# Autodesk Inventor assembly: Plattenzusammensetzung
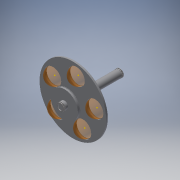
[picture p0: Inventor's stored thumbnail of the model, 180x180]
Saved by Autodesk Inventor 2016 (Build 200138000, 138)
## iProperties
Created: 2017-10-13
Part Number: Plattenzusammensetzung
Material: Generisch
Document SubType Name: Assembly
Designer: Dominik
Author: Dominik
## Documents named in this file (6)
- C:\Users\Dominik\Desktop\Diplomarbeit\Inverntorskizzen\Plattenzusammensetzung.iam
- C:\Users\Dominik\Desktop\Diplomarbeit\Inverntorskizzen\Antriebsscheibe.ipt
- C:\Users\Dominik\Desktop\Diplomarbeit\Inverntorskizzen\Drehplatte_Rahmenvorrrichtung.ipt
- C:\Users\Dominik\Desktop\Diplomarbeit\Inverntorskizzen\Futterschüssel_innen.ipt
- C:\Users\Dominik\Desktop\Diplomarbeit\Inverntorskizzen\Welle.ipt
- C:\Users\Dominik\Documents\Inventor\Content Center Files\R2016\de-DE\DIN 711\DIN 711 - 511 06 - 30 x 47 x 11.ipt
## Components (10 placed, 5 different names)
1. Antriebsscheibe:1 — Passend:2
2. Drehplatte_Rahmenvorrrichtung:1 — Passend:1, Passend:3, Passend:4, Passend:5, Passend:6, Passend:7, Passend:8, Passend:9, Passend:10, Passend:11, Passend:12
3. Futterschüssel_innen:1 — Passend:3, Passend:4
4. Welle:1 — Passend:1, Passend:2, Passend:13, Passend:14, Passend:15, Passend:16
5. Futterschüssel_innen:2 — Passend:5, Passend:6
6. Futterschüssel_innen:3 — Passend:11, Passend:12
7. Futterschüssel_innen:4 — Passend:9, Passend:10
8. Futterschüssel_innen:5 — Passend:7, Passend:8
9. DIN 711 511 06 - 30 x 47 x 11:1 — Passend:13, Passend:16
10. DIN 711 511 06 - 30 x 47 x 11:2 — Passend:14, Passend:15
## Relationships (16: Mate 16)
- Passend:1 [Mate]: Drehplatte_Rahmenvorrrichtung:1 ↔ Welle:1
- Passend:2 [Mate]: Antriebsscheibe:1 ↔ Welle:1
- Passend:3 [Mate]: Drehplatte_Rahmenvorrrichtung:1 ↔ Futterschüssel_innen:1
- Passend:4 [Mate]: Drehplatte_Rahmenvorrrichtung:1 ↔ Futterschüssel_innen:1
- Passend:5 [Mate]: Drehplatte_Rahmenvorrrichtung:1 ↔ Futterschüssel_innen:2
- Passend:6 [Mate]: Drehplatte_Rahmenvorrrichtung:1 ↔ Futterschüssel_innen:2
- Passend:7 [Mate]: Drehplatte_Rahmenvorrrichtung:1 ↔ Futterschüssel_innen:5
- Passend:8 [Mate]: Drehplatte_Rahmenvorrrichtung:1 ↔ Futterschüssel_innen:5
- Passend:9 [Mate]: Drehplatte_Rahmenvorrrichtung:1 ↔ Futterschüssel_innen:4
- Passend:10 [Mate]: Drehplatte_Rahmenvorrrichtung:1 ↔ Futterschüssel_innen:4
- Passend:11 [Mate]: Drehplatte_Rahmenvorrrichtung:1 ↔ Futterschüssel_innen:3
- Passend:12 [Mate]: Drehplatte_Rahmenvorrrichtung:1 ↔ Futterschüssel_innen:3
- Passend:13 [Mate]: Welle:1 ↔ DIN 711 511 06 - 30 x 47 x 11:1
- Passend:14 [Mate]: Welle:1 ↔ DIN 711 511 06 - 30 x 47 x 11:2
- Passend:15 [Mate]: Welle:1 ↔ DIN 711 511 06 - 30 x 47 x 11:2
- Passend:16 [Mate]: Welle:1 ↔ DIN 711 511 06 - 30 x 47 x 11:1
